# Autodesk Inventor assembly: Cablecar
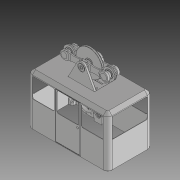
[picture p0: Inventor's stored thumbnail of the model, 180x180]
Saved by Autodesk Inventor 2020 (Build 240168000, 168)
## iProperties
Created: 2021-02-03
Part Number: Cablecar
Document SubType Name: Assembly
Designer: DDeGo
Author: DDeGo
## Documents named in this file (10)
- C:\Users\DDeGo\Documents\Drew\Projects\AirWankelEngine\cad\Cablecar\Cablecar.iam
- C:\Users\DDeGo\Documents\Drew\Projects\AirWankelEngine\cad\Cablecar\Cablecar_frame.ipt
- C:\Users\DDeGo\Documents\Drew\Projects\AirWankelEngine\cad\Cablecar\Cablecar_topbracket.ipt
- C:\Users\DDeGo\Documents\Drew\Projects\AirWankelEngine\cad\hardware\625 Bearing.ipt
- C:\Users\DDeGo\Documents\Drew\Projects\AirWankelEngine\cad\Cablecar\Cablecar_drivepulley.ipt
- C:\Users\DDeGo\Documents\Drew\Projects\AirWankelEngine\cad\Cablecar\Cablecar_pulleybracket.ipt
- C:\Users\DDeGo\Documents\Drew\Projects\AirWankelEngine\cad\hardware\6701 bearing.ipt
- C:\Users\DDeGo\Documents\Drew\Projects\AirWankelEngine\cad\Cablecar\Cablecar_idlepulley.ipt
- C:\Users\DDeGo\Documents\Drew\Projects\AirWankelEngine\cad\Cablecar\Cablecar_spacer.ipt
- C:\Users\DDeGo\Documents\Drew\Projects\AirWankelEngine\cad\EngineAssembly.iam
## Components (19 placed, 9 different names)
1. Cablecar_frame:1 — Mate:1, Mate:2, Mate:3, Mate:32, Mate:33, Mate:34
2. Cablecar_topbracket:1 — Mate:1, Mate:2, Mate:3, Mate:4, Mate:5, Flush:1, Flush:2
3. 625 Bearing:1 — Mate:4, Flush:2, Mate:6, Mate:8
4. 625 Bearing:2 — Mate:5, Flush:1, Mate:7, Mate:9
5. Cablecar_drivepulley:1 — Mate:10, Flush:5, Flush:6, Mate:18
6. Cablecar_pulleybracket:1 — Mate:7, Mate:9, Mate:12, Mate:15, Mate:16, Mate:17, Mate:23
7. Cablecar_pulleybracket:2 — Mate:6, Mate:8, Mate:17
8. 6701 bearing:1 — Mate:10, Mate:12, Mate:18, Mate:26, Mate:27, Mate:30, Mate:31
9. Cablecar_idlepulley:1 — Mate:13, Flush:3, Flush:5
10. 6701 bearing:2 — Mate:13, Flush:3, Mate:15, Mate:24, Mate:25, Mate:28, Mate:29
11. Cablecar_idlepulley:2 — Flush:6
12. 6701 bearing:3 — Mate:16, Mate:19, Mate:20, Mate:21, Mate:22
13. Cablecar_spacer:1 — Mate:19, Mate:20
14. Cablecar_spacer:2 — Mate:21, Mate:22, Mate:23
15. Cablecar_spacer:3 — Mate:26, Mate:30
16. Cablecar_spacer:4 — Mate:25, Mate:28
17. Cablecar_spacer:5 — Mate:24, Mate:29
18. Cablecar_spacer:6 — Mate:27, Mate:31
19. EngineAssembly:1 [sub-assembly] — Mate:32, Mate:33, Mate:34
## Relationships (39: Mate 33, Flush 6)
- Mate:1: Cablecar_frame:1 ↔ Cablecar_topbracket:1
- Mate:2: Cablecar_frame:1 ↔ Cablecar_topbracket:1
- Mate:3: Cablecar_frame:1 ↔ Cablecar_topbracket:1
- Mate:4: Cablecar_topbracket:1 ↔ 625 Bearing:1
- Mate:5: Cablecar_topbracket:1 ↔ 625 Bearing:2
- Flush:1: Cablecar_topbracket:1 ↔ 625 Bearing:2
- Flush:2: Cablecar_topbracket:1 ↔ 625 Bearing:1
- Mate:6: 625 Bearing:1 ↔ Cablecar_pulleybracket:2
- Mate:7: 625 Bearing:2 ↔ Cablecar_pulleybracket:1
- Mate:8: 625 Bearing:1 ↔ Cablecar_pulleybracket:2
- Mate:9: 625 Bearing:2 ↔ Cablecar_pulleybracket:1
- Mate:10: Cablecar_drivepulley:1 ↔ 6701 bearing:1
- Mate:12: Cablecar_pulleybracket:1 ↔ 6701 bearing:1
- Mate:13: Cablecar_idlepulley:1 ↔ 6701 bearing:2
- Flush:3: Cablecar_idlepulley:1 ↔ 6701 bearing:2
- [Mate]: Cablecar_idlepulley:2 ↔ 6701 bearing:3
- [Flush]: Cablecar_idlepulley:2 ↔ 6701 bearing:3
- Mate:15: Cablecar_pulleybracket:1 ↔ 6701 bearing:2
- Mate:16: Cablecar_pulleybracket:1 ↔ 6701 bearing:3
- Mate:17: Cablecar_pulleybracket:1 ↔ Cablecar_pulleybracket:2
- Flush:5: Cablecar_drivepulley:1 ↔ Cablecar_idlepulley:1
- Flush:6: Cablecar_drivepulley:1 ↔ Cablecar_idlepulley:2
- Mate:18: Cablecar_drivepulley:1 ↔ 6701 bearing:1
- Mate:19: 6701 bearing:3 ↔ Cablecar_spacer:1
- Mate:20: 6701 bearing:3 ↔ Cablecar_spacer:1
- Mate:21: 6701 bearing:3 ↔ Cablecar_spacer:2
- Mate:22: 6701 bearing:3 ↔ Cablecar_spacer:2
- Mate:23: Cablecar_pulleybracket:1 ↔ Cablecar_spacer:2
- Mate:24: 6701 bearing:2 ↔ Cablecar_spacer:5
- Mate:25: 6701 bearing:2 ↔ Cablecar_spacer:4
- Mate:26: 6701 bearing:1 ↔ Cablecar_spacer:3
- Mate:27: 6701 bearing:1 ↔ Cablecar_spacer:6
- Mate:28: 6701 bearing:2 ↔ Cablecar_spacer:4
- Mate:29: 6701 bearing:2 ↔ Cablecar_spacer:5
- Mate:30: 6701 bearing:1 ↔ Cablecar_spacer:3
- Mate:31: 6701 bearing:1 ↔ Cablecar_spacer:6
- Mate:32: Cablecar_frame:1 ↔ EngineAssembly:1
- Mate:33: Cablecar_frame:1 ↔ EngineAssembly:1
- Mate:34: Cablecar_frame:1 ↔ EngineAssembly:1
## Named parameters: d16_d14 = 0 mm, d17_d15 = 0 mm
